# Autodesk Inventor assembly: hinge flag
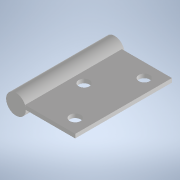
[picture p0: Inventor's stored thumbnail of the model, 180x180]
Saved by Autodesk Inventor 2020 (Build 240168000, 168)
## iProperties
Created: 2023-04-24
Part Number: hinge flag
Document SubType Name: Assembly
Designer: super
Author: super
## Documents named in this file (3)
- C:\desk\promissionsave\inventor\robot\hinge flag.iam
- C:\desk\promissionsave\inventor\robot\hinge flag plate.ipt
- C:\desk\promissionsave\inventor\robot\hinge cilinder.ipt
## Components (2 placed, 2 different names)
1. hinge flag plate:2 — Flush:1
2. hinge cilinder:1 — Flush:1
## Relationships (1: Flush 1)
- Flush:1: hinge flag plate:2 ↔ hinge cilinder:1
